# Autodesk Inventor assembly: haptic_ass_1
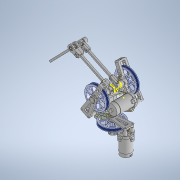
[picture p0: Inventor's stored thumbnail of the model, 180x180]
Saved by Autodesk Inventor 2020 (Build 240168000, 168)
## iProperties
Created: 2019-10-15
Part Number: haptic_ass_1
Document SubType Name: Assembly
Designer: psrob
Author: psrob
## Documents named in this file (14)
- E:\projects-2\haptic device gen3\hardware\export_20191015\haptic_ass_1.iam
- E:\projects-2\haptic device gen3\hardware\upper_arm_1.iam
- E:\projects-2\haptic device gen3\hardware\belt_reducer_2.iam
- E:\projects-2\haptic device gen3\hardware\export_20191015\armtip_1.ipt
- E:\projects-2\haptic device gen3\hardware\armtip_2.ipt
- E:\projects-2\haptic device gen3\hardware\carbon_fiber_1.ipt
- E:\projects-2\haptic device gen3\hardware\export_20191015\armtip_3.ipt
- E:\projects-2\haptic device gen3\hardware\bearing_6_13_5.ipt
- E:\projects-2\haptic device gen3\hardware\sub_arm_1.ipt
- E:\projects-2\haptic device gen3\hardware\sub_arm_2.ipt
- E:\projects-2\haptic device gen3\hardware\arm_linkage_1.ipt
- E:\projects-2\haptic device gen3\hardware\bearing_3_10_5.ipt
- E:\projects-2\haptic device gen3\hardware\arm_linkage_2.ipt
- E:\projects-2\haptic device gen3\hardware\arm_linkage_3.ipt
## Components (22 placed, 13 different names)
1. upper_arm_1:1 [sub-assembly] — Insert:1, Insert:2, Insert:3, Insert:13
2. belt_reducer_2:1 [sub-assembly] — Insert:1, Insert:2
3. armtip_1:1 — Insert:3, Mate:1, Mate:2, Mate:3, Insert:4, Insert:5
4. armtip_2:1 — Insert:4, Insert:5
5. carbon_fiber_1:1 — Mate:1, Mate:2, Mate:3, Mate:4, Mate:5, Mate:6
6. armtip_3:1 — Insert:6, Insert:7, Insert:8
7. armtip_3:2 — Mate:4, Mate:5, Mate:6, Insert:6, Insert:7, Insert:9
8. bearing_6_13_5:1 — Insert:8, Insert:24
9. bearing_6_13_5:2 — Insert:9
10. sub_arm_1:1 — Mate:7, Mate:8, Mate:9, Flush:2, Insert:11, Insert:12, Insert:14, Insert:15, Insert:24
11. carbon_fiber_1:2 — Mate:7, Mate:8, Mate:9
12. sub_arm_2:1 — Flush:2, Insert:11, Insert:12, Angle:1
13. arm_linkage_1:1 — Insert:13, Insert:16, Insert:17, Angle:1
14. bearing_3_10_5:1 — Insert:14
15. bearing_3_10_5:2 — Insert:15
16. bearing_3_10_5:3 — Insert:16, Insert:19
17. bearing_3_10_5:4 — Insert:17
18. arm_linkage_2:1 — Mate:10, Mate:11, Mate:12, Insert:22, Insert:23
19. arm_linkage_2:2 — Insert:19, Mate:13, Mate:14, Flush:4, Insert:20, Insert:21
20. carbon_fiber_1:3 — Mate:10, Mate:11, Mate:12, Mate:13, Mate:14, Mate:15
21. arm_linkage_3:1 — Flush:4, Insert:20, Insert:21, Mate:15
22. arm_linkage_3:2 — Insert:22, Insert:23
## Relationships (40: Insert 22, Mate 15, Flush 2, Angle 1)
- Insert:1: upper_arm_1:1 ↔ belt_reducer_2:1
- Insert:2: upper_arm_1:1 ↔ belt_reducer_2:1
- Insert:3: upper_arm_1:1 ↔ armtip_1:1
- Mate:1: armtip_1:1 ↔ carbon_fiber_1:1
- Mate:2: armtip_1:1 ↔ carbon_fiber_1:1
- Mate:3: armtip_1:1 ↔ carbon_fiber_1:1
- Insert:4: armtip_1:1 ↔ armtip_2:1
- Insert:5: armtip_1:1 ↔ armtip_2:1
- Mate:4: carbon_fiber_1:1 ↔ armtip_3:2
- Mate:5: carbon_fiber_1:1 ↔ armtip_3:2
- Mate:6: carbon_fiber_1:1 ↔ armtip_3:2
- Insert:6: armtip_3:1 ↔ armtip_3:2
- Insert:7: armtip_3:1 ↔ armtip_3:2
- Insert:8: armtip_3:1 ↔ bearing_6_13_5:1
- Insert:9: armtip_3:2 ↔ bearing_6_13_5:2
- Mate:7: sub_arm_1:1 ↔ carbon_fiber_1:2
- Mate:8: sub_arm_1:1 ↔ carbon_fiber_1:2
- Mate:9: sub_arm_1:1 ↔ carbon_fiber_1:2
- Flush:2: sub_arm_1:1 ↔ sub_arm_2:1
- Insert:11: sub_arm_1:1 ↔ sub_arm_2:1
- Insert:12: sub_arm_1:1 ↔ sub_arm_2:1
- Insert:13 (-5 mm): upper_arm_1:1 ↔ arm_linkage_1:1
- Insert:14: sub_arm_1:1 ↔ bearing_3_10_5:1
- Insert:15: sub_arm_1:1 ↔ bearing_3_10_5:2
- Insert:16: arm_linkage_1:1 ↔ bearing_3_10_5:3
- Insert:17: arm_linkage_1:1 ↔ bearing_3_10_5:4
- Angle:1 (0 deg): sub_arm_2:1 ↔ arm_linkage_1:1
- Insert:19: bearing_3_10_5:3 ↔ arm_linkage_2:2
- Mate:10: arm_linkage_2:1 ↔ carbon_fiber_1:3
- Mate:11: arm_linkage_2:1 ↔ carbon_fiber_1:3
- Mate:12: arm_linkage_2:1 ↔ carbon_fiber_1:3
- Mate:13: arm_linkage_2:2 ↔ carbon_fiber_1:3
- Mate:14: arm_linkage_2:2 ↔ carbon_fiber_1:3
- Flush:4: arm_linkage_2:2 ↔ arm_linkage_3:1
- Insert:20: arm_linkage_2:2 ↔ arm_linkage_3:1
- Insert:21: arm_linkage_2:2 ↔ arm_linkage_3:1
- Insert:22: arm_linkage_2:1 ↔ arm_linkage_3:2
- Insert:23: arm_linkage_2:1 ↔ arm_linkage_3:2
- Insert:24: bearing_6_13_5:1 ↔ sub_arm_1:1
- Mate:15: carbon_fiber_1:3 ↔ arm_linkage_3:1
